# Autodesk Inventor assembly: Ensamble_completo
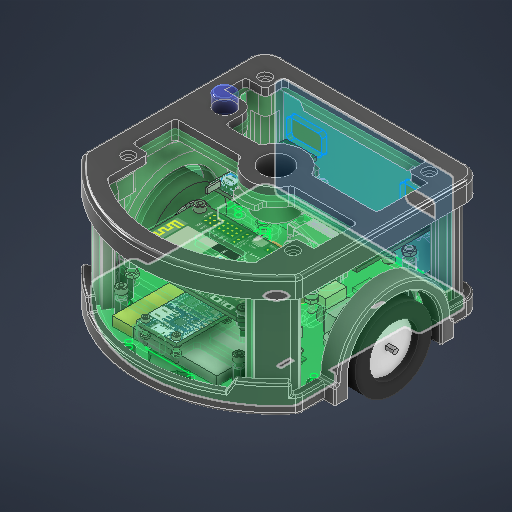
[picture p0: Inventor's stored thumbnail of the model, 512x512]
Saved by Autodesk Inventor 2026 (Build 300175000, 175)
## iProperties
Created: 2025-10-21
Part Number: Ensamble_completo
Document SubType Name: Assembly
Designer: brene
Author: brene
## Documents named in this file (44)
- C:\Users\aavalerin\Documents\GitSHit\Atta-Bot-STEM\Chasis\Diseño V3.0\Ensamble_completo.iam
- C:\Users\aavalerin\Documents\GitSHit\Atta-Bot-STEM\Chasis\Diseño V3.0\base_chasis_v6\base_chasis_v4-dimsAjustadas.ipt
- C:\Users\aavalerin\Documents\GitSHit\Atta-Bot-STEM\Chasis\Diseño V3.0\base_chasis_v6.ipt
- C:\Users\aavalerin\Documents\GitSHit\Atta-Bot-STEM\Chasis\Diseño V3.0\Content Center Files\en-US\ISO 4762(2)\ISO 4762 - M2 x 12ISO.ipt
- C:\Users\aavalerin\Documents\GitSHit\Atta-Bot-STEM\Chasis\Diseño V3.0\switch.ipt
- C:\Users\aavalerin\Documents\GitSHit\Atta-Bot-STEM\Chasis\Diseño V3.0\Content Center Files\en-US\ISO 4762(2)\ISO 4762 - M2 x 8ISO.ipt
- C:\Users\aavalerin\Documents\GitSHit\Atta-Bot-STEM\Chasis\Diseño V3.0\Content Center Files\en-US\ISO 4032(2)\ISO 4032 - M2 - ISO.ipt
- C:\Users\aavalerin\Documents\GitSHit\Atta-Bot-STEM\Chasis\Diseño V3.0\ball_caster.ipt
- C:\Users\aavalerin\Documents\GitSHit\Atta-Bot-STEM\Chasis\Diseño V3.0\sensorInferior.ipt
- C:\Users\aavalerin\Documents\GitSHit\Atta-Bot-STEM\Chasis\Diseño V3.0\Content Center Files\en-US\ISO 4762(2)\ISO 4762 - M3 x 12ISO.ipt
- C:\Users\aavalerin\Documents\GitSHit\Atta-Bot-STEM\Chasis\Diseño V3.0\Content Center Files\en-US\ISO 4032(2)\ISO 4032 - M3 - ISO.ipt
- C:\Users\aavalerin\Documents\GitSHit\Atta-Bot-STEM\Chasis\Diseño V3.0\spacers\hexagonal_spacer_MF_M3_H20_HEX5.5_FTD6_MTL6.ipt
- C:\Users\aavalerin\Documents\GitSHit\Atta-Bot-STEM\Chasis\Diseño V3.0\spacers\hexagonal_spacer_MF_M3_H06_HEX5.5_FTD3_MTL6.ipt
- C:\Users\aavalerin\Documents\GitSHit\Atta-Bot-STEM\Chasis\Diseño V3.0\Content Center Files\en-US\ISO 4762(2)\ISO 4762 - M3 x 8ISO.ipt
- C:\Users\aavalerin\Documents\GitSHit\Atta-Bot-STEM\Chasis\Diseño V3.0\spacers\hexagonal_spacer_MF_M3_H08_HEX5_FTD4_MTL8.ipt
- C:\Users\aavalerin\Documents\GitSHit\Atta-Bot-STEM\Chasis\Diseño V3.0\bateria.ipt
- C:\Users\aavalerin\Documents\GitSHit\Atta-Bot-STEM\Chasis\Diseño V3.0\base_powerboost.ipt
- C:\Users\aavalerin\Documents\GitSHit\Atta-Bot-STEM\Chasis\Diseño V3.0\powerboost.ipt
- C:\Users\aavalerin\Documents\GitSHit\Atta-Bot-STEM\Chasis\Diseño V3.0\base_nivel2.ipt
- C:\Users\aavalerin\Documents\GitSHit\Atta-Bot-STEM\Chasis\Diseño V3.0\ideaboard.ipt
- C:\Users\aavalerin\Documents\GitSHit\Atta-Bot-STEM\Chasis\Diseño V3.0\sensorFrontal.ipt
- C:\Users\aavalerin\Documents\GitSHit\Atta-Bot-STEM\Chasis\Diseño V3.0\Tower Pro MG90S Micro servo.ipt
- C:\Users\aavalerin\Documents\GitSHit\Atta-Bot-STEM\Chasis\Diseño V3.0\spacers\hexagonal_spacer_MF_M3_H10_HEX5.5_FTD6_MTL6.ipt
- C:\Users\aavalerin\Documents\GitSHit\Atta-Bot-STEM\Chasis\Diseño V3.0\SoporteMotor_3.0.ipt
- C:\Users\aavalerin\Documents\GitSHit\Atta-Bot-STEM\Chasis\Diseño V3.0\motor.ipt
- C:\Users\aavalerin\Documents\GitSHit\Atta-Bot-STEM\Chasis\Diseño V3.0\llanta.ipt
- C:\Users\aavalerin\Documents\GitSHit\Atta-Bot-STEM\Chasis\Diseño V3.0\Unidirectional shoulder.ipt
- C:\Users\aavalerin\Documents\GitSHit\Atta-Bot-STEM\Chasis\Diseño V3.0\SujecionServo.ipt
- C:\Users\aavalerin\Documents\GitSHit\Atta-Bot-STEM\Chasis\Diseño V3.0\PrensaPilotAttaBotStem\PrensaPilotAttaBotStem\PrensaPilotAttaBotStem.ipt
- C:\Users\06aar\Documents\Inventor\Content Center Files\R2026\en-US\SS-ISO 4762\ISO 4762 - M2,5 x 25SS-ISO.ipt
- C:\Users\aavalerin\Documents\GitSHit\Atta-Bot-STEM\Chasis\Diseño V3.0\Esquinero Trasero\base_chasis_v4-dimsAjustadas.ipt
- C:\Users\aavalerin\Documents\GitSHit\Atta-Bot-STEM\Chasis\Diseño V3.0\Esquinero Trasero.ipt
- C:\Users\aavalerin\Documents\GitSHit\Atta-Bot-STEM\Chasis\Diseño V3.0\Bumper Trasero\base_chasis_v4-dimsAjustadas.ipt
- C:\Users\aavalerin\Documents\GitSHit\Atta-Bot-STEM\Chasis\Diseño V3.0\Bumper Trasero.ipt
- C:\Users\aavalerin\Documents\GitSHit\Atta-Bot-STEM\Chasis\Diseño V3.0\Guardabarros.ipt
- C:\Users\aavalerin\Documents\GitSHit\Atta-Bot-STEM\Chasis\Diseño V3.0\Bumper Delantero.ipt
- C:\Users\aavalerin\Documents\GitSHit\Atta-Bot-STEM\Chasis\Diseño V3.0\Esquineros Delanteros.ipt
- C:\Users\aavalerin\Documents\GitSHit\Atta-Bot-STEM\Chasis\Diseño V3.0\PARED TRASERA.ipt
- C:\Users\aavalerin\Documents\GitSHit\Atta-Bot-STEM\Chasis\Diseño V3.0\PAREDES LATERALES.ipt
- C:\Users\aavalerin\Documents\GitSHit\Atta-Bot-STEM\Chasis\Diseño V3.0\PAREDES LATERALES_MIR.ipt
- C:\Users\aavalerin\Documents\GitSHit\Atta-Bot-STEM\Chasis\Diseño V3.0\PARED FRONTAL.ipt
- C:\Users\aavalerin\Documents\GitSHit\Atta-Bot-STEM\Chasis\Diseño V3.0\Techo Armadura.ipt
- C:\Users\aavalerin\Documents\GitSHit\Atta-Bot-STEM\Chasis\Diseño V3.0\Acrilicos Superiores.ipt
- C:\Users\aavalerin\Documents\GitSHit\Atta-Bot-STEM\Chasis\Diseño V3.0\Pieza de Silicona.ipt
## Components (118 placed, 38 different names)
1. Pieza de Silicona:1 — Flush:213, Mate:268
2. Guardabarros:1 — Mate:270, Mate:272, Mate:273
3. hexagonal_spacer_MF_M3_H10_HEX5.5_FTD6_MTL6:4 — Mate:212, Mate:216, Mate:220, Mate:221
4. hexagonal_spacer_MF_M3_H10_HEX5.5_FTD6_MTL6:3 — Mate:211, Angle:8, Mate:218, Mate:219
5. ISO 4762 M3 x 8:10 — Mate:151, Mate:152
6. ISO 4762 M3 x 8:9 — Mate:153, Mate:154
7. hexagonal_spacer_MF_M3_H10_HEX5.5_FTD6_MTL6:2 — Mate:148, Mate:150
8. hexagonal_spacer_MF_M3_H10_HEX5.5_FTD6_MTL6:1 — Mate:147, Mate:149
9. ISO 4762 M3 x 8:8 — Mate:113, Mate:114, Mate:250, Mate:251
10. ISO 4762 M3 x 8:7 — Mate:117, Mate:118
11. ISO 4032 M3:8 — Mate:123, Mate:124
12. ISO 4032 M3:7 — Mate:125, Mate:126
13. hexagonal_spacer_MF_M3_H06_HEX5.5_FTD3_MTL6:10 — Mate:115, Mate:116, Mate:119, Mate:120, Mate:126
14. hexagonal_spacer_MF_M3_H06_HEX5.5_FTD3_MTL6:9 — Mate:111, Mate:112, Mate:121, Mate:122, Mate:124
15. hexagonal_spacer_MF_M3_H06_HEX5.5_FTD3_MTL6:8 — Mate:104, Mate:105, Mate:108, Mate:110, Mate:132, Mate:175
16. hexagonal_spacer_MF_M3_H06_HEX5.5_FTD3_MTL6:7 — Mate:106, Mate:107, Mate:134, Mate:177
17. hexagonal_spacer_MF_M3_H06_HEX5.5_FTD3_MTL6:6 — Mate:100, Mate:101, Mate:109, Mate:130, Mate:179, Mate:275, Mate:276, Mate:277, Mate:278, Mate:279, Mate:280, Mate:281
18. hexagonal_spacer_MF_M3_H06_HEX5.5_FTD3_MTL6:5 — Mate:102, Mate:103, Mate:128, Mate:181
19. ISO 4762 M3 x 8:6 — Mate:94, Mate:95
20. ISO 4762 M3 x 8:5 — Mate:96, Mate:97
21. ISO 4762 M3 x 8:4 — Mate:92, Mate:93
22. ISO 4762 M3 x 8:3 — Mate:98, Mate:99
23. ISO 4032 M2:10 — Mate:84, Mate:85
24. ISO 4032 M2:9 — Mate:80, Mate:81
25. ISO 4032 M2:8 — Mate:86, Mate:87
26. ISO 4032 M2:7 — Mate:82, Mate:83
27. ISO 4032 M2:6 — Mate:64, Mate:65, Mate:70
28. ISO 4032 M2:5 — Mate:66, Mate:67
29. ISO 4032 M2:4 — Mate:62, Mate:63, Mate:71
30. ISO 4032 M2:3 — Mate:68, Mate:69
31. ISO 4762 M2 x 8:6 — Mate:76, Mate:77, Mate:87, Mate:91
32. ISO 4762 M2 x 8:5 — Mate:78, Mate:79, Mate:85
33. ISO 4762 M2 x 12:2 — Mate:72, Mate:73, Mate:83
34. ISO 4762 M2 x 12:1 — Mate:74, Mate:75, Mate:81
35. ISO 4032 M3:6 — Mate:48, Mate:49, Mate:57
36. ISO 4032 M3:5 — Mate:50, Mate:51, Mate:59
37. ISO 4032 M3:4 — Mate:46, Mate:47, Mate:53
38. ISO 4032 M3:3 — Mate:44, Mate:45, Mate:55
39. hexagonal_spacer_MF_M3_H08_HEX5_FTD4_MTL8:4 — Mate:54, Mate:55, Mate:90
40. hexagonal_spacer_MF_M3_H08_HEX5_FTD4_MTL8:3 — Mate:52, Mate:53, Mate:89
41. hexagonal_spacer_MF_M3_H08_HEX5_FTD4_MTL8:2 — Mate:58, Mate:59, Mate:88
42. hexagonal_spacer_MF_M3_H08_HEX5_FTD4_MTL8:1 — Mate:56, Mate:57, Mate:61
43. ISO 4762 M3 x 8:2 — Mate:34, Mate:35, Mate:39
44. ISO 4762 M3 x 8:1 — Mate:32, Mate:33, Mate:37
45. hexagonal_spacer_MF_M3_H20_HEX5.5_FTD6_MTL6:4 — Mate:36, Mate:37, Mate:137, Mate:145
46. hexagonal_spacer_MF_M3_H20_HEX5.5_FTD6_MTL6:3 — Mate:38, Mate:39, Mate:143
47. hexagonal_spacer_MF_M3_H20_HEX5.5_FTD6_MTL6:2 — Mate:26, Mate:27, Mate:135, Mate:141
48. hexagonal_spacer_MF_M3_H20_HEX5.5_FTD6_MTL6:1 — Mate:24, Mate:25, Mate:136, Mate:139
49. ISO 4032 M3:2 — Mate:14, Mate:15, Mate:18, Mate:19, Mate:23
50. ISO 4032 M3:1 — Mate:12, Mate:13, Mate:16, Mate:17, Mate:21
51. ISO 4762 M3 x 12:2 — Mate:22, Mate:23, Mate:27
52. ISO 4762 M3 x 12:1 — Mate:20, Mate:21, Mate:25
53. ISO 4762 M2 x 8:4 — Mate:8, Mate:9, Tangent:4
54. ISO 4762 M2 x 8:3 — Mate:10, Mate:11, Tangent:3
55. ISO 4032 M2:2 — Insert:2
56. ISO 4032 M2:1 — Insert:1
57. ISO 4762 M2 x 8:2 — Mate:3, Mate:4
58. ISO 4762 M2 x 8:1 — Mate:5, Mate:6
59. ISO 4032 M3:16 — Mate:144, Mate:145
60. ISO 4032 M3:15 — Mate:140, Mate:141
61. ISO 4032 M3:14 — Mate:138, Mate:139
62. ISO 4032 M3:13 — Mate:142, Mate:143
63. ISO 4032 M3:12 — Mate:127, Mate:128
64. ISO 4032 M3:11 — Mate:131, Mate:132
65. ISO 4032 M3:10 — Mate:129, Mate:130
66. ISO 4032 M3:9 — Mate:133, Mate:134
67. ISO 4032 M2:15 — Mate:194, Mate:195
68. ISO 4032 M2:14 — Mate:196, Mate:197
69. ISO 4032 M2:13 — Mate:192, Mate:193
70. ISO 4032 M2:12 — Mate:190, Mate:191
71. ISO 4762 M2 x 8:10 — Mate:183, Mate:197
72. ISO 4762 M2 x 8:9 — Mate:187, Mate:193
73. ISO 4762 M2 x 8:8 — Mate:189, Mate:191
74. ISO 4762 M2 x 8:7 — Mate:185, Mate:195
75. ISO 4762 M3 x 8:14 — Mate:174, Mate:175
76. ISO 4762 M3 x 8:13 — Mate:178, Mate:179
77. ISO 4762 M3 x 8:12 — Mate:180, Mate:181, Mate:274
78. ISO 4762 M3 x 8:11 — Mate:176, Mate:177
79. SS ISO 4762 M2,5 x 25:13 — Insert:19
80. SS ISO 4762 M2,5 x 25:12 — Insert:18
81. SS ISO 4762 M2,5 x 25:11 — Insert:17
82. SS ISO 4762 M2,5 x 25:9 — Insert:15
83. SS ISO 4762 M2,5 x 25:8 — Insert:14
84. SS ISO 4762 M2,5 x 25:6 — Insert:12
85. SS ISO 4762 M2,5 x 25:4 — Insert:10
86. SS ISO 4762 M2,5 x 25:1 — Insert:7
87. switch:1 — Mate:1, Mate:2, Mate:3, Mate:5, Angle:3
88. ball_caster:1 — Mate:7, Tangent:1, Tangent:2, Mate:9, Mate:11
89. sensorInferior:1 — Mate:16, Mate:17, Mate:20, Angle:7
90. bateria:1 — Mate:60, Mate:61, Mate:146, Angle:2
91. sensorInferior:2 — Mate:18, Mate:19, Mate:22, Angle:6
92. base_powerboost:1 — Mate:62, Mate:63, Mate:64, Mate:65, Mate:66, Mate:67, Mate:68, Mate:69, Mate:80, Mate:82, Mate:84, Mate:86, Mate:88, Mate:89, Mate:90, Mate:91, Mate:92, Mate:93, Mate:94, Mate:95, Mate:96, Mate:97, Mate:98, Mate:99
93. powerboost:1 — Mate:70, Mate:71, Mate:72, Mate:73, Mate:74, Mate:75, Mate:76, Mate:77, Mate:78, Mate:79
94. base_nivel2:1 — Mate:100, Mate:101, Mate:102, Mate:103, Mate:104, Mate:105, Mate:106, Mate:107, Mate:111, Mate:112, Mate:113, Mate:114, Mate:115, Mate:116, Mate:117, Mate:118, Mate:127, Mate:129, Mate:131, Mate:133, Mate:135, Mate:136, Mate:137, Mate:138, Mate:140, Mate:142, Mate:144, Angle:4, Angle:5, Mate:250, Mate:251, Mate:274, Mate:275, Mate:276, Mate:277, Mate:278, Mate:279, Mate:280, Mate:281
95. ideaboard:1 — Mate:108, Mate:109, Mate:110, Mate:174, Mate:176, Mate:178, Mate:180
96. sensorFrontal:1 — Mate:121, Mate:122, Mate:123, Angle:5
97. motor:1 — Mate:161, Mate:163, Mate:164, Mate:227, Tangent:5
98. sensorFrontal:2 — Mate:119, Mate:120, Mate:125, Angle:4
99. motor:2 — Mate:169, Mate:171, Mate:172, Mate:230, Tangent:6
100. llanta:1 — Mate:163, Mate:164, Mate:272
101. llanta:2 — Mate:171, Mate:172
102. Tower Pro MG90S Micro servo:2 — Mate:205, Mate:206, Mate:207, Angle:1, Angle:8, Mate:217, Mate:221
103. Unidirectional shoulder:1 — Mate:205, Mate:206
104. SujecionServo:1 — Mate:216, Mate:217, Mate:219
105. SoporteMotor_3.0:1 — Mate:229, Mate:230, Mate:231, Mate:233, Tangent:6
106. SoporteMotor_3.0:2 — Mate:226, Mate:227, Mate:228, Tangent:5, Mate:232
107. PARED TRASERA:1 — Mate:253, Mate:254
108. PAREDES LATERALES:2 — Mate:255, Mate:256, Mate:257
109. PAREDES LATERALES_MIR:1
110. PARED FRONTAL:1 — Mate:258, Mate:259, Mate:260, Mate:269
111. Acrilicos Superiores:1 — Mate:265, Mate:266, Mate:267
112. base_chasis_v4-dimsAjustadas:3 — Flush:212, Mate:237, Mate:238, Mate:256, Mate:261, Mate:263, Mate:264
113. base_chasis_v4-dimsAjustadas:1 — Mate:239, Mate:240, Mate:244, Mate:254
114. base_chasis_v4-dimsAjustadas:2 — Mate:1, Mate:2, Mate:4, Mate:6, Insert:1, Insert:2, Mate:7, Tangent:1, Tangent:2, Mate:8, Mate:10, Tangent:3, Tangent:4, Mate:12, Mate:13, Mate:14, Mate:15, Mate:24, Mate:26, Mate:32, Mate:33, Mate:34, Mate:35, Mate:36, Mate:38, Mate:44, Mate:45, Mate:46, Mate:47, Mate:48, Mate:49, Mate:50, Mate:51, Mate:52, Mate:54, Mate:56, Mate:58, Mate:60, Mate:146, Mate:147, Mate:148, Mate:149, Mate:150, Mate:151, Mate:152, Mate:153, Mate:154, Mate:161, Mate:169, Mate:183, Mate:185, Mate:187, Mate:189, Mate:190, Mate:192, Mate:194, Mate:196, Mate:207, Angle:1, Mate:209, Flush:211, Mate:210, Angle:2, Angle:3, Angle:6, Angle:7, Mate:211, Mate:212, Mate:218, Mate:220, Mate:226, Mate:228, Mate:229, Mate:231, Mate:232, Mate:233, Mate:234, Mate:235, Mate:236, Insert:7, Insert:10, Insert:12, Insert:14, Insert:15, Insert:17, Insert:18, Insert:19, Flush:212, Mate:237, Mate:238, Mate:239, Mate:240, Mate:244, Mate:245, Mate:246, Mate:247, Mate:249, Mate:253, Mate:255, Mate:258, Mate:262, Mate:270, Mate:273
115. PrensaPilotAttaBotStem:1 — Mate:234, Mate:235, Mate:236
116. Bumper Delantero:1 — Mate:245, Mate:246, Mate:247, Mate:248, Mate:252, Mate:259
117. Esquineros Delanteros:1 — Mate:248, Mate:249, Mate:252, Mate:257, Mate:260, Mate:269
118. Techo Armadura:1 — Mate:261, Mate:262, Mate:263, Mate:264, Mate:265, Mate:266, Mate:267, Flush:213, Mate:268
## Relationships (264: Mate 237, Insert 10, Angle 8, Tangent 6, Flush 3)
- Mate:1: switch:1 ↔ base_chasis_v4-dimsAjustadas:2
- Mate:2: switch:1 ↔ base_chasis_v4-dimsAjustadas:2
- Mate:3: ISO 4762 M2 x 8:2 ↔ switch:1
- Mate:4: ISO 4762 M2 x 8:2 ↔ base_chasis_v4-dimsAjustadas:2
- Mate:5: ISO 4762 M2 x 8:1 ↔ switch:1
- Mate:6: ISO 4762 M2 x 8:1 ↔ base_chasis_v4-dimsAjustadas:2
- Insert:1: ISO 4032 M2:1 ↔ base_chasis_v4-dimsAjustadas:2
- Insert:2: ISO 4032 M2:2 ↔ base_chasis_v4-dimsAjustadas:2
- Mate:7: ball_caster:1 ↔ base_chasis_v4-dimsAjustadas:2
- Tangent:1: ball_caster:1 ↔ base_chasis_v4-dimsAjustadas:2
- Tangent:2: ball_caster:1 ↔ base_chasis_v4-dimsAjustadas:2
- Mate:8: ISO 4762 M2 x 8:4 ↔ base_chasis_v4-dimsAjustadas:2
- Mate:9: ISO 4762 M2 x 8:4 ↔ ball_caster:1
- Mate:10: ISO 4762 M2 x 8:3 ↔ base_chasis_v4-dimsAjustadas:2
- Mate:11: ISO 4762 M2 x 8:3 ↔ ball_caster:1
- Tangent:3: ISO 4762 M2 x 8:3 ↔ base_chasis_v4-dimsAjustadas:2
- Tangent:4: ISO 4762 M2 x 8:4 ↔ base_chasis_v4-dimsAjustadas:2
- Mate:12: ISO 4032 M3:1 ↔ base_chasis_v4-dimsAjustadas:2
- Mate:13: ISO 4032 M3:1 ↔ base_chasis_v4-dimsAjustadas:2
- Mate:14: ISO 4032 M3:2 ↔ base_chasis_v4-dimsAjustadas:2
- Mate:15: ISO 4032 M3:2 ↔ base_chasis_v4-dimsAjustadas:2
- Mate:16: ISO 4032 M3:1 ↔ sensorInferior:1
- Mate:17: ISO 4032 M3:1 ↔ sensorInferior:1
- Mate:18: ISO 4032 M3:2 ↔ sensorInferior:2
- Mate:19: ISO 4032 M3:2 ↔ sensorInferior:2
- Mate:20: ISO 4762 M3 x 12:1 ↔ sensorInferior:1
- Mate:21: ISO 4032 M3:1 ↔ ISO 4762 M3 x 12:1
- Mate:22: ISO 4762 M3 x 12:2 ↔ sensorInferior:2
- Mate:23: ISO 4032 M3:2 ↔ ISO 4762 M3 x 12:2
- Mate:24: hexagonal_spacer_MF_M3_H20_HEX5.5_FTD6_MTL6:1 ↔ base_chasis_v4-dimsAjustadas:2
- Mate:25: hexagonal_spacer_MF_M3_H20_HEX5.5_FTD6_MTL6:1 ↔ ISO 4762 M3 x 12:1
- Mate:26: hexagonal_spacer_MF_M3_H20_HEX5.5_FTD6_MTL6:2 ↔ base_chasis_v4-dimsAjustadas:2
- Mate:27: hexagonal_spacer_MF_M3_H20_HEX5.5_FTD6_MTL6:2 ↔ ISO 4762 M3 x 12:2
- Mate:32: ISO 4762 M3 x 8:1 ↔ base_chasis_v4-dimsAjustadas:2
- Mate:33: ISO 4762 M3 x 8:1 ↔ base_chasis_v4-dimsAjustadas:2
- Mate:34: ISO 4762 M3 x 8:2 ↔ base_chasis_v4-dimsAjustadas:2
- Mate:35: ISO 4762 M3 x 8:2 ↔ base_chasis_v4-dimsAjustadas:2
- Mate:36: hexagonal_spacer_MF_M3_H20_HEX5.5_FTD6_MTL6:4 ↔ base_chasis_v4-dimsAjustadas:2
- Mate:37: ISO 4762 M3 x 8:1 ↔ hexagonal_spacer_MF_M3_H20_HEX5.5_FTD6_MTL6:4
- Mate:38: hexagonal_spacer_MF_M3_H20_HEX5.5_FTD6_MTL6:3 ↔ base_chasis_v4-dimsAjustadas:2
- Mate:39: ISO 4762 M3 x 8:2 ↔ hexagonal_spacer_MF_M3_H20_HEX5.5_FTD6_MTL6:3
- Mate:44: ISO 4032 M3:3 ↔ base_chasis_v4-dimsAjustadas:2
- Mate:45: ISO 4032 M3:3 ↔ base_chasis_v4-dimsAjustadas:2
- Mate:46: ISO 4032 M3:4 ↔ base_chasis_v4-dimsAjustadas:2
- Mate:47: ISO 4032 M3:4 ↔ base_chasis_v4-dimsAjustadas:2
- Mate:48: ISO 4032 M3:6 ↔ base_chasis_v4-dimsAjustadas:2
- Mate:49: ISO 4032 M3:6 ↔ base_chasis_v4-dimsAjustadas:2
- Mate:50: ISO 4032 M3:5 ↔ base_chasis_v4-dimsAjustadas:2
- Mate:51: ISO 4032 M3:5 ↔ base_chasis_v4-dimsAjustadas:2
- Mate:52: hexagonal_spacer_MF_M3_H08_HEX5_FTD4_MTL8:3 ↔ base_chasis_v4-dimsAjustadas:2
- Mate:53: ISO 4032 M3:4 ↔ hexagonal_spacer_MF_M3_H08_HEX5_FTD4_MTL8:3
- Mate:54: hexagonal_spacer_MF_M3_H08_HEX5_FTD4_MTL8:4 ↔ base_chasis_v4-dimsAjustadas:2
- Mate:55: ISO 4032 M3:3 ↔ hexagonal_spacer_MF_M3_H08_HEX5_FTD4_MTL8:4
- Mate:56: hexagonal_spacer_MF_M3_H08_HEX5_FTD4_MTL8:1 ↔ base_chasis_v4-dimsAjustadas:2
- Mate:57: ISO 4032 M3:6 ↔ hexagonal_spacer_MF_M3_H08_HEX5_FTD4_MTL8:1
- Mate:58: hexagonal_spacer_MF_M3_H08_HEX5_FTD4_MTL8:2 ↔ base_chasis_v4-dimsAjustadas:2
- Mate:59: ISO 4032 M3:5 ↔ hexagonal_spacer_MF_M3_H08_HEX5_FTD4_MTL8:2
- Mate:60: bateria:1 ↔ base_chasis_v4-dimsAjustadas:2
- Mate:61: hexagonal_spacer_MF_M3_H08_HEX5_FTD4_MTL8:1 ↔ bateria:1
- Mate:62: ISO 4032 M2:4 ↔ base_powerboost:1
- Mate:63: ISO 4032 M2:4 ↔ base_powerboost:1
- Mate:64: ISO 4032 M2:6 ↔ base_powerboost:1
- Mate:65: ISO 4032 M2:6 ↔ base_powerboost:1
- Mate:66: ISO 4032 M2:5 ↔ base_powerboost:1
- Mate:67: ISO 4032 M2:5 ↔ base_powerboost:1
- Mate:68: ISO 4032 M2:3 ↔ base_powerboost:1
- Mate:69: ISO 4032 M2:3 ↔ base_powerboost:1
- Mate:70: ISO 4032 M2:6 ↔ powerboost:1
- Mate:71: ISO 4032 M2:4 ↔ powerboost:1
- Mate:72: ISO 4762 M2 x 12:2 ↔ powerboost:1
- Mate:73: ISO 4762 M2 x 12:2 ↔ powerboost:1
- Mate:74: ISO 4762 M2 x 12:1 ↔ powerboost:1
- Mate:75: ISO 4762 M2 x 12:1 ↔ powerboost:1
- Mate:76: ISO 4762 M2 x 8:6 ↔ powerboost:1
- Mate:77: ISO 4762 M2 x 8:6 ↔ powerboost:1
- Mate:78: ISO 4762 M2 x 8:5 ↔ powerboost:1
- Mate:79: ISO 4762 M2 x 8:5 ↔ powerboost:1
- Mate:80: ISO 4032 M2:9 ↔ base_powerboost:1
- Mate:81: ISO 4032 M2:9 ↔ ISO 4762 M2 x 12:1
- Mate:82: ISO 4032 M2:7 ↔ base_powerboost:1
- Mate:83: ISO 4032 M2:7 ↔ ISO 4762 M2 x 12:2
- Mate:84: ISO 4032 M2:10 ↔ base_powerboost:1
- Mate:85: ISO 4032 M2:10 ↔ ISO 4762 M2 x 8:5
- Mate:86: ISO 4032 M2:8 ↔ base_powerboost:1
- Mate:87: ISO 4032 M2:8 ↔ ISO 4762 M2 x 8:6
- Mate:88: hexagonal_spacer_MF_M3_H08_HEX5_FTD4_MTL8:2 ↔ base_powerboost:1
- Mate:89: hexagonal_spacer_MF_M3_H08_HEX5_FTD4_MTL8:3 ↔ base_powerboost:1
- Mate:90: hexagonal_spacer_MF_M3_H08_HEX5_FTD4_MTL8:4 ↔ base_powerboost:1
- Mate:91: ISO 4762 M2 x 8:6 ↔ base_powerboost:1
- Mate:92: ISO 4762 M3 x 8:4 ↔ base_powerboost:1
- Mate:93: ISO 4762 M3 x 8:4 ↔ base_powerboost:1
- Mate:94: ISO 4762 M3 x 8:6 ↔ base_powerboost:1
- Mate:95: ISO 4762 M3 x 8:6 ↔ base_powerboost:1
- Mate:96: ISO 4762 M3 x 8:5 ↔ base_powerboost:1
- Mate:97: ISO 4762 M3 x 8:5 ↔ base_powerboost:1
- Mate:98: ISO 4762 M3 x 8:3 ↔ base_powerboost:1
- Mate:99: ISO 4762 M3 x 8:3 ↔ base_powerboost:1
- Mate:100: hexagonal_spacer_MF_M3_H06_HEX5.5_FTD3_MTL6:6 ↔ base_nivel2:1
- Mate:101: hexagonal_spacer_MF_M3_H06_HEX5.5_FTD3_MTL6:6 ↔ base_nivel2:1
- Mate:102: hexagonal_spacer_MF_M3_H06_HEX5.5_FTD3_MTL6:5 ↔ base_nivel2:1
- Mate:103: hexagonal_spacer_MF_M3_H06_HEX5.5_FTD3_MTL6:5 ↔ base_nivel2:1
- Mate:104: hexagonal_spacer_MF_M3_H06_HEX5.5_FTD3_MTL6:8 ↔ base_nivel2:1
- Mate:105: hexagonal_spacer_MF_M3_H06_HEX5.5_FTD3_MTL6:8 ↔ base_nivel2:1
- Mate:106: hexagonal_spacer_MF_M3_H06_HEX5.5_FTD3_MTL6:7 ↔ base_nivel2:1
- Mate:107: hexagonal_spacer_MF_M3_H06_HEX5.5_FTD3_MTL6:7 ↔ base_nivel2:1
- Mate:108: hexagonal_spacer_MF_M3_H06_HEX5.5_FTD3_MTL6:8 ↔ ideaboard:1
- Mate:109: hexagonal_spacer_MF_M3_H06_HEX5.5_FTD3_MTL6:6 ↔ ideaboard:1
- Mate:110: hexagonal_spacer_MF_M3_H06_HEX5.5_FTD3_MTL6:8 ↔ ideaboard:1
- Mate:111: hexagonal_spacer_MF_M3_H06_HEX5.5_FTD3_MTL6:9 ↔ base_nivel2:1
- Mate:112: hexagonal_spacer_MF_M3_H06_HEX5.5_FTD3_MTL6:9 ↔ base_nivel2:1
- Mate:113: ISO 4762 M3 x 8:8 ↔ base_nivel2:1
- Mate:114: ISO 4762 M3 x 8:8 ↔ base_nivel2:1
- Mate:115: hexagonal_spacer_MF_M3_H06_HEX5.5_FTD3_MTL6:10 ↔ base_nivel2:1
- Mate:116: hexagonal_spacer_MF_M3_H06_HEX5.5_FTD3_MTL6:10 ↔ base_nivel2:1
- Mate:117: ISO 4762 M3 x 8:7 ↔ base_nivel2:1
- Mate:118: ISO 4762 M3 x 8:7 ↔ base_nivel2:1
- Mate:119: hexagonal_spacer_MF_M3_H06_HEX5.5_FTD3_MTL6:10 ↔ sensorFrontal:2
- Mate:120: hexagonal_spacer_MF_M3_H06_HEX5.5_FTD3_MTL6:10 ↔ sensorFrontal:2
- Mate:121: hexagonal_spacer_MF_M3_H06_HEX5.5_FTD3_MTL6:9 ↔ sensorFrontal:1
- Mate:122: hexagonal_spacer_MF_M3_H06_HEX5.5_FTD3_MTL6:9 ↔ sensorFrontal:1
- Mate:123: ISO 4032 M3:8 ↔ sensorFrontal:1
- Mate:124: ISO 4032 M3:8 ↔ hexagonal_spacer_MF_M3_H06_HEX5.5_FTD3_MTL6:9
- Mate:125: ISO 4032 M3:7 ↔ sensorFrontal:2
- Mate:126: ISO 4032 M3:7 ↔ hexagonal_spacer_MF_M3_H06_HEX5.5_FTD3_MTL6:10
- Mate:127: ISO 4032 M3:12 ↔ base_nivel2:1
- Mate:128: hexagonal_spacer_MF_M3_H06_HEX5.5_FTD3_MTL6:5 ↔ ISO 4032 M3:12
- Mate:129: ISO 4032 M3:10 ↔ base_nivel2:1
- Mate:130: hexagonal_spacer_MF_M3_H06_HEX5.5_FTD3_MTL6:6 ↔ ISO 4032 M3:10
- Mate:131: ISO 4032 M3:11 ↔ base_nivel2:1
- Mate:132: hexagonal_spacer_MF_M3_H06_HEX5.5_FTD3_MTL6:8 ↔ ISO 4032 M3:11
- Mate:133: ISO 4032 M3:9 ↔ base_nivel2:1
- Mate:134: hexagonal_spacer_MF_M3_H06_HEX5.5_FTD3_MTL6:7 ↔ ISO 4032 M3:9
- Mate:135: hexagonal_spacer_MF_M3_H20_HEX5.5_FTD6_MTL6:2 ↔ base_nivel2:1
- Mate:136: hexagonal_spacer_MF_M3_H20_HEX5.5_FTD6_MTL6:1 ↔ base_nivel2:1
- Mate:137: hexagonal_spacer_MF_M3_H20_HEX5.5_FTD6_MTL6:4 ↔ base_nivel2:1
- Mate:138: ISO 4032 M3:14 ↔ base_nivel2:1
- Mate:139: hexagonal_spacer_MF_M3_H20_HEX5.5_FTD6_MTL6:1 ↔ ISO 4032 M3:14
- Mate:140: ISO 4032 M3:15 ↔ base_nivel2:1
- Mate:141: hexagonal_spacer_MF_M3_H20_HEX5.5_FTD6_MTL6:2 ↔ ISO 4032 M3:15
- Mate:142: ISO 4032 M3:13 ↔ base_nivel2:1
- Mate:143: hexagonal_spacer_MF_M3_H20_HEX5.5_FTD6_MTL6:3 ↔ ISO 4032 M3:13
- Mate:144: ISO 4032 M3:16 ↔ base_nivel2:1
- Mate:145: hexagonal_spacer_MF_M3_H20_HEX5.5_FTD6_MTL6:4 ↔ ISO 4032 M3:16
- Mate:146: bateria:1 ↔ base_chasis_v4-dimsAjustadas:2
- Mate:147: hexagonal_spacer_MF_M3_H10_HEX5.5_FTD6_MTL6:1 ↔ base_chasis_v4-dimsAjustadas:2
- Mate:148: hexagonal_spacer_MF_M3_H10_HEX5.5_FTD6_MTL6:2 ↔ base_chasis_v4-dimsAjustadas:2
- Mate:149: hexagonal_spacer_MF_M3_H10_HEX5.5_FTD6_MTL6:1 ↔ base_chasis_v4-dimsAjustadas:2
- Mate:150: hexagonal_spacer_MF_M3_H10_HEX5.5_FTD6_MTL6:2 ↔ base_chasis_v4-dimsAjustadas:2
- Mate:151: ISO 4762 M3 x 8:10 ↔ base_chasis_v4-dimsAjustadas:2
- Mate:152: ISO 4762 M3 x 8:10 ↔ base_chasis_v4-dimsAjustadas:2
- Mate:153: ISO 4762 M3 x 8:9 ↔ base_chasis_v4-dimsAjustadas:2
- Mate:154: ISO 4762 M3 x 8:9 ↔ base_chasis_v4-dimsAjustadas:2
- Mate:161: motor:1 ↔ base_chasis_v4-dimsAjustadas:2
- Mate:163: motor:1 ↔ llanta:1
- Mate:164: motor:1 ↔ llanta:1
- Mate:169: motor:2 ↔ base_chasis_v4-dimsAjustadas:2
- Mate:171: motor:2 ↔ llanta:2
- Mate:172: motor:2 ↔ llanta:2
- Mate:174: ISO 4762 M3 x 8:14 ↔ ideaboard:1
- Mate:175: hexagonal_spacer_MF_M3_H06_HEX5.5_FTD3_MTL6:8 ↔ ISO 4762 M3 x 8:14
- Mate:176: ISO 4762 M3 x 8:11 ↔ ideaboard:1
- Mate:177: hexagonal_spacer_MF_M3_H06_HEX5.5_FTD3_MTL6:7 ↔ ISO 4762 M3 x 8:11
- Mate:178: ISO 4762 M3 x 8:13 ↔ ideaboard:1
- Mate:179: hexagonal_spacer_MF_M3_H06_HEX5.5_FTD3_MTL6:6 ↔ ISO 4762 M3 x 8:13
- Mate:180: ISO 4762 M3 x 8:12 ↔ ideaboard:1
- Mate:181: hexagonal_spacer_MF_M3_H06_HEX5.5_FTD3_MTL6:5 ↔ ISO 4762 M3 x 8:12
- Mate:183: ISO 4762 M2 x 8:10 ↔ base_chasis_v4-dimsAjustadas:2
- Mate:185: ISO 4762 M2 x 8:7 ↔ base_chasis_v4-dimsAjustadas:2
- Mate:187: ISO 4762 M2 x 8:9 ↔ base_chasis_v4-dimsAjustadas:2
- Mate:189: ISO 4762 M2 x 8:8 ↔ base_chasis_v4-dimsAjustadas:2
- Mate:190: ISO 4032 M2:12 ↔ base_chasis_v4-dimsAjustadas:2
- Mate:191: ISO 4032 M2:12 ↔ ISO 4762 M2 x 8:8
- Mate:192: ISO 4032 M2:13 ↔ base_chasis_v4-dimsAjustadas:2
- Mate:193: ISO 4032 M2:13 ↔ ISO 4762 M2 x 8:9
- Mate:194: ISO 4032 M2:15 ↔ base_chasis_v4-dimsAjustadas:2
- Mate:195: ISO 4032 M2:15 ↔ ISO 4762 M2 x 8:7
- Mate:196: ISO 4032 M2:14 ↔ base_chasis_v4-dimsAjustadas:2
- Mate:197: ISO 4032 M2:14 ↔ ISO 4762 M2 x 8:10
- Mate:205: Tower Pro MG90S Micro servo:2 ↔ Unidirectional shoulder:1
- Mate:206 (1 mm): Tower Pro MG90S Micro servo:2 ↔ Unidirectional shoulder:1
- Mate:207: Tower Pro MG90S Micro servo:2 ↔ base_chasis_v4-dimsAjustadas:2
- Angle:1 (0 deg): Tower Pro MG90S Micro servo:2 ↔ base_chasis_v4-dimsAjustadas:2
- Mate:209: base_chasis_v4-dimsAjustadas:2
- Flush:211: base_chasis_v4-dimsAjustadas:2
- Mate:210: base_chasis_v4-dimsAjustadas:2
- Angle:2 (0 deg): bateria:1 ↔ base_chasis_v4-dimsAjustadas:2
- Angle:3 (180 deg): switch:1 ↔ base_chasis_v4-dimsAjustadas:2
- Angle:4 (180 deg): base_nivel2:1 ↔ sensorFrontal:2
- Angle:5 (180 deg): base_nivel2:1 ↔ sensorFrontal:1
- Angle:6 (180 deg): sensorInferior:2 ↔ base_chasis_v4-dimsAjustadas:2
- Angle:7 (180 deg): sensorInferior:1 ↔ base_chasis_v4-dimsAjustadas:2
- Mate:211: hexagonal_spacer_MF_M3_H10_HEX5.5_FTD6_MTL6:3 ↔ base_chasis_v4-dimsAjustadas:2
- Mate:212: hexagonal_spacer_MF_M3_H10_HEX5.5_FTD6_MTL6:4 ↔ base_chasis_v4-dimsAjustadas:2
- Angle:8 (-90 deg): hexagonal_spacer_MF_M3_H10_HEX5.5_FTD6_MTL6:3 ↔ Tower Pro MG90S Micro servo:2
- Mate:216: hexagonal_spacer_MF_M3_H10_HEX5.5_FTD6_MTL6:4 ↔ SujecionServo:1
- Mate:217: Tower Pro MG90S Micro servo:2 ↔ SujecionServo:1
- Mate:218: hexagonal_spacer_MF_M3_H10_HEX5.5_FTD6_MTL6:3 ↔ base_chasis_v4-dimsAjustadas:2
- Mate:219: hexagonal_spacer_MF_M3_H10_HEX5.5_FTD6_MTL6:3 ↔ SujecionServo:1
- Mate:220: hexagonal_spacer_MF_M3_H10_HEX5.5_FTD6_MTL6:4 ↔ base_chasis_v4-dimsAjustadas:2
- Mate:221: hexagonal_spacer_MF_M3_H10_HEX5.5_FTD6_MTL6:4 ↔ Tower Pro MG90S Micro servo:2
- Mate:226: SoporteMotor_3.0:2 ↔ base_chasis_v4-dimsAjustadas:2
- Mate:227: motor:1 ↔ SoporteMotor_3.0:2
- Mate:228: SoporteMotor_3.0:2 ↔ base_chasis_v4-dimsAjustadas:2
- Mate:229: SoporteMotor_3.0:1 ↔ base_chasis_v4-dimsAjustadas:2
- Mate:230: motor:2 ↔ SoporteMotor_3.0:1
- Mate:231: SoporteMotor_3.0:1 ↔ base_chasis_v4-dimsAjustadas:2
- Tangent:5: motor:1 ↔ SoporteMotor_3.0:2
- Mate:232: SoporteMotor_3.0:2 ↔ base_chasis_v4-dimsAjustadas:2
- Mate:233: SoporteMotor_3.0:1 ↔ base_chasis_v4-dimsAjustadas:2
- Tangent:6: motor:2 ↔ SoporteMotor_3.0:1
- Mate:234: base_chasis_v4-dimsAjustadas:2 ↔ PrensaPilotAttaBotStem:1
- Mate:235: base_chasis_v4-dimsAjustadas:2 ↔ PrensaPilotAttaBotStem:1
- Mate:236: base_chasis_v4-dimsAjustadas:2 ↔ PrensaPilotAttaBotStem:1
- Insert:7: SS ISO 4762 M2,5 x 25:1 ↔ base_chasis_v4-dimsAjustadas:2
- Insert:10: SS ISO 4762 M2,5 x 25:4 ↔ base_chasis_v4-dimsAjustadas:2
- Insert:12: SS ISO 4762 M2,5 x 25:6 ↔ base_chasis_v4-dimsAjustadas:2
- Insert:14: SS ISO 4762 M2,5 x 25:8 ↔ base_chasis_v4-dimsAjustadas:2
- Insert:15: SS ISO 4762 M2,5 x 25:9 ↔ base_chasis_v4-dimsAjustadas:2
- Insert:17: SS ISO 4762 M2,5 x 25:11 ↔ base_chasis_v4-dimsAjustadas:2
- Insert:18: SS ISO 4762 M2,5 x 25:12 ↔ base_chasis_v4-dimsAjustadas:2
- Insert:19: SS ISO 4762 M2,5 x 25:13 ↔ base_chasis_v4-dimsAjustadas:2
- Flush:212: base_chasis_v4-dimsAjustadas:3 ↔ base_chasis_v4-dimsAjustadas:2
- Mate:237: base_chasis_v4-dimsAjustadas:3 ↔ base_chasis_v4-dimsAjustadas:2
- Mate:238: base_chasis_v4-dimsAjustadas:3 ↔ base_chasis_v4-dimsAjustadas:2
- Mate:239: base_chasis_v4-dimsAjustadas:1 ↔ base_chasis_v4-dimsAjustadas:2
- Mate:240: base_chasis_v4-dimsAjustadas:1 ↔ base_chasis_v4-dimsAjustadas:2
- Mate:244: base_chasis_v4-dimsAjustadas:1 ↔ base_chasis_v4-dimsAjustadas:2
- Mate:245: base_chasis_v4-dimsAjustadas:2 ↔ Bumper Delantero:1
- Mate:246: base_chasis_v4-dimsAjustadas:2 ↔ Bumper Delantero:1
- Mate:247: base_chasis_v4-dimsAjustadas:2 ↔ Bumper Delantero:1
- Mate:248: Bumper Delantero:1 ↔ Esquineros Delanteros:1
- Mate:249: base_chasis_v4-dimsAjustadas:2 ↔ Esquineros Delanteros:1
- Mate:250: ISO 4762 M3 x 8:8 ↔ base_nivel2:1
- Mate:251: ISO 4762 M3 x 8:8 ↔ base_nivel2:1
- Mate:252: Bumper Delantero:1 ↔ Esquineros Delanteros:1
- Mate:253: PARED TRASERA:1 ↔ base_chasis_v4-dimsAjustadas:2
- Mate:254: PARED TRASERA:1 ↔ base_chasis_v4-dimsAjustadas:1
- Mate:255: PAREDES LATERALES:2 ↔ base_chasis_v4-dimsAjustadas:2
- Mate:256: PAREDES LATERALES:2 ↔ base_chasis_v4-dimsAjustadas:3
- Mate:257: PAREDES LATERALES:2 ↔ Esquineros Delanteros:1
- Mate:258: PARED FRONTAL:1 ↔ base_chasis_v4-dimsAjustadas:2
- Mate:259: PARED FRONTAL:1 ↔ Bumper Delantero:1
- Mate:260: PARED FRONTAL:1 ↔ Esquineros Delanteros:1
- Mate:261: base_chasis_v4-dimsAjustadas:3 ↔ Techo Armadura:1
- Mate:262: base_chasis_v4-dimsAjustadas:2 ↔ Techo Armadura:1
- Mate:263: base_chasis_v4-dimsAjustadas:3 ↔ Techo Armadura:1
- Mate:264: base_chasis_v4-dimsAjustadas:3 ↔ Techo Armadura:1
- Mate:265: Acrilicos Superiores:1 ↔ Techo Armadura:1
- Mate:266: Acrilicos Superiores:1 ↔ Techo Armadura:1
- Mate:267: Acrilicos Superiores:1 ↔ Techo Armadura:1
- Flush:213: Pieza de Silicona:1 ↔ Techo Armadura:1
- Mate:268: Pieza de Silicona:1 ↔ Techo Armadura:1
- Mate:269: PARED FRONTAL:1 ↔ Esquineros Delanteros:1
- Mate:270: Guardabarros:1 ↔ base_chasis_v4-dimsAjustadas:2
- Mate:272: Guardabarros:1 ↔ llanta:1
- Mate:273: Guardabarros:1 ↔ base_chasis_v4-dimsAjustadas:2
- Mate:274: ISO 4762 M3 x 8:12 ↔ base_nivel2:1
- Mate:275: hexagonal_spacer_MF_M3_H06_HEX5.5_FTD3_MTL6:6 ↔ base_nivel2:1
- Mate:276: hexagonal_spacer_MF_M3_H06_HEX5.5_FTD3_MTL6:6 ↔ base_nivel2:1
- Mate:277: hexagonal_spacer_MF_M3_H06_HEX5.5_FTD3_MTL6:6 ↔ base_nivel2:1
- Mate:278: hexagonal_spacer_MF_M3_H06_HEX5.5_FTD3_MTL6:6 ↔ base_nivel2:1
- Mate:279: hexagonal_spacer_MF_M3_H06_HEX5.5_FTD3_MTL6:6 ↔ base_nivel2:1
- Mate:280: hexagonal_spacer_MF_M3_H06_HEX5.5_FTD3_MTL6:6 ↔ base_nivel2:1
- Mate:281: hexagonal_spacer_MF_M3_H06_HEX5.5_FTD3_MTL6:6 ↔ base_nivel2:1
